# Autodesk Inventor assembly: SpMax_Drive
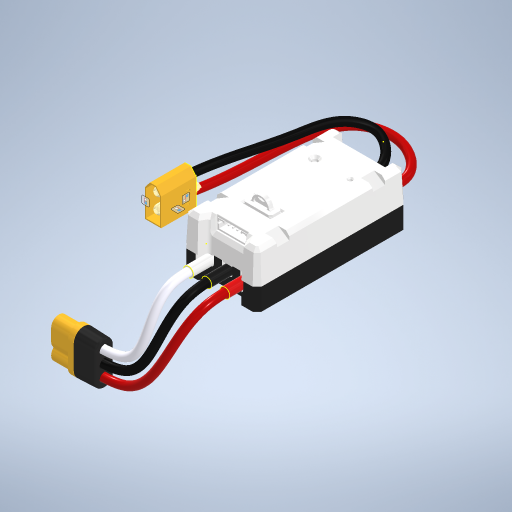
[picture p0: Inventor's stored thumbnail of the model, 512x512]
Saved by Autodesk Inventor 2023.4 (Build 274418000, 418)
## iProperties
Created: 2023-09-14
Part Number: SpMax_Drive
Document SubType Name: Assembly
Designer: adamarnold
Author: adamarnold
## Documents named in this file (4)
- G:\.shortcut-targets-by-id\104lhnwPhYvankLacu8RGROV89Bx_24Mg\1939\2_Design\2023-2024\Parts\Electronics\SpMax_Drive.iam
- G:\.shortcut-targets-by-id\104lhnwPhYvankLacu8RGROV89Bx_24Mg\1939\2_Design\2023-2024\Parts\Electronics\REV-11-2158-Spark-MAX_Wired.ipt
- G:\.shortcut-targets-by-id\104lhnwPhYvankLacu8RGROV89Bx_24Mg\1939\2_Design\2023-2024\Parts\Electronics\Component Wiring\SPM_Power_Phase_Wiring.iam
- G:\.shortcut-targets-by-id\104lhnwPhYvankLacu8RGROV89Bx_24Mg\1939\2_Design\2023-2024\Parts\Electronics\Connectors\MR60_Plug.iam
## Components (3 placed, 3 different names)
1. REV-11-2158-Spark-MAX_Wired:1 — Mate:1, Flush:1, Mate:2, Mate:4, Flush:4, Mate:5
2. MR60_Plug:1 [sub-assembly] — Mate:4, Flush:4, Mate:5
3. SPM_Power_Phase_Wiring [sub-assembly]
## Relationships (9: Mate 5, Flush 4)
- Mate:1: REV-11-2158-Spark-MAX_Wired:1
- Flush:1: REV-11-2158-Spark-MAX_Wired:1
- Mate:2: REV-11-2158-Spark-MAX_Wired:1
- [Flush] (12.7 mm): REV-11-2158-Spark-MAX_Wired:1 ↔ SPM_Power_Phase_Wiring
- [Flush]: REV-11-2158-Spark-MAX_Wired:1 ↔ SPM_Power_Phase_Wiring
- [Mate] (9.525 mm): REV-11-2158-Spark-MAX_Wired:1 ↔ SPM_Power_Phase_Wiring
- Mate:4 (16.0274 mm): REV-11-2158-Spark-MAX_Wired:1 ↔ MR60_Plug:1
- Flush:4 (66.294 mm): REV-11-2158-Spark-MAX_Wired:1 ↔ MR60_Plug:1
- Mate:5 (38.1 mm): REV-11-2158-Spark-MAX_Wired:1 ↔ MR60_Plug:1
